# Autodesk Inventor assembly: ElectronicsLayout
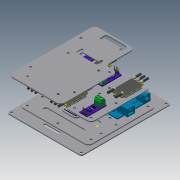
[picture p0: Inventor's stored thumbnail of the model, 180x180]
Saved by Autodesk Inventor 2018 (Build 220112000, 112)
## iProperties
Created: 2019-03-24
Part Number: ElectronicsLayout
Document SubType Name: Assembly
Designer: anirudh
Author: anirudh
## Documents named in this file (14)
- D:\Silicon Sharks\2018-2019\ElectronicsHousing\Electronics Layout\ElectronicsLayout.iam
- D:\Silicon Sharks\2018-2019\ElectronicsHousing\Electronics Layout\Tier1Plate.ipt
- C:\Users\anirudh\Documents\MARS Fund\MATE Robotics\Silicon Sharks\2018-2019\ElectronicsHousing\Electronics Layout\Hex Spacer MF M3 L6mm.ipt
- C:\Users\anirudh\Documents\MARS Fund\MATE Robotics\Silicon Sharks\2018-2019\ElectronicsHousing\Electronics Layout\Hex Spacer MF M3 L20mm.ipt
- D:\Silicon Sharks\2018-2019\ElectronicsHousing\Electronics Layout\Tier2Plate.ipt
- D:\Silicon Sharks\2018-2019\ElectronicsHousing\Electronics Layout\BESC30-R3.ipt
- D:\Silicon Sharks\2018-2019\ElectronicsHousing\Electronics Layout\ACS 712 Stromsensor für Arduino.ipt
- D:\Silicon Sharks\2018-2019\ElectronicsHousing\Electronics Layout\Tier3Plate.ipt
- D:\Silicon Sharks\2018-2019\ElectronicsHousing\Electronics Layout\PCB2x8.ipt
- D:\Silicon Sharks\2018-2019\ElectronicsHousing\Electronics Layout\ArduinoMega_STEP_AP203.ipt
- D:\Silicon Sharks\2018-2019\ElectronicsHousing\Electronics Layout\Tier4.ipt
- D:\Silicon Sharks\2018-2019\ElectronicsHousing\Electronics Layout\Adafruit_BNO055_AP214.ipt
- C:\Users\anirudh\Documents\MARS Fund\MATE Robotics\Silicon Sharks\2018-2019\ElectronicsHousing\Electronics Layout\Hex Spacer MF M3 L8mm.ipt
- D:\Silicon Sharks\2018-2019\ElectronicsHousing\Electronics Layout\Tier5.ipt
## Components (40 placed, 13 different names)
1. Tier1Plate:1 — Mate:1, Mate:2, Mate:3, Mate:4, Mate:5, Mate:6, Mate:7, Mate:8, Mate:9, Mate:10, Mate:11, Mate:12, Mate:13, Mate:14, Mate:15, Mate:16, Mate:17, Mate:18, Mate:19, Mate:20, Mate:21, Mate:22, Mate:23, Mate:24
2. Hex Spacer MF M3 L6mm:1 — Mate:1, Mate:12
3. Hex Spacer MF M3 L6mm:2 — Mate:2, Mate:13
4. Hex Spacer MF M3 L6mm:3 — Mate:4, Mate:11
5. Hex Spacer MF M3 L6mm:4 — Mate:3, Mate:14
6. Hex Spacer MF M3 L6mm:5 — Mate:7, Mate:15
7. Hex Spacer MF M3 L6mm:6 — Mate:8, Mate:9
8. Hex Spacer MF M3 L6mm:7 — Mate:5, Mate:16
9. Hex Spacer MF M3 L6mm:8 — Mate:6, Mate:10
10. Hex Spacer MF M3 L20mm:1 — Mate:18, Mate:21, Mate:26
11. Hex Spacer MF M3 L20mm:2 — Mate:17, Mate:22, Mate:25, Mate:27
12. Hex Spacer MF M3 L20mm:3 — Mate:19, Mate:23
13. Hex Spacer MF M3 L20mm:4 — Mate:20, Mate:24
14. Tier2Plate:1 — Mate:25, Mate:26, Mate:27, Mate:28, Mate:29, Mate:30, Mate:31, Mate:32, Mate:33, Mate:34, Mate:35, Mate:36, Mate:37, Mate:38, Mate:39, Flush:3, Flush:4, Flush:5, Flush:6, Flush:7, Flush:8, Flush:9, Flush:10, Flush:11, Flush:12, Flush:13, Flush:14, Flush:15, Flush:16, Flush:17, Flush:18, Mate:93, Mate:94, Mate:95
15. BESC30-R3:1 — Mate:28, Flush:5, Flush:6
16. BESC30-R3:2 — Mate:29, Flush:3, Flush:4
17. BESC30-R3:3 — Mate:30, Flush:7, Flush:8
18. BESC30-R3:4 — Mate:31, Flush:9, Flush:10
19. ACS 712 Stromsensor für Arduino:1 — Mate:33, Flush:15, Flush:17
20. ACS 712 Stromsensor für Arduino:2 — Mate:35, Flush:11, Flush:12
21. ACS 712 Stromsensor für Arduino:3 — Mate:32, Flush:16, Flush:18
22. ACS 712 Stromsensor für Arduino:4 — Mate:34, Flush:13, Flush:14
23. Hex Spacer MF M3 L6mm:9 — Mate:36, Mate:39, Mate:40, Mate:42
24. Hex Spacer MF M3 L6mm:10 — Mate:37, Mate:38, Mate:41
25. Tier3Plate:1 — Mate:40, Mate:41, Mate:42, Flush:1, Flush:2, Mate:43, Mate:64, Mate:65, Mate:66
26. PCB2x8:1 — Flush:1, Flush:2, Mate:43
27. Adafruit_BNO055_AP214:1 — Mate:64, Mate:65, Mate:66
28. Tier4:1 — Mate:67, Mate:68, Mate:69, Mate:70, Mate:71, Mate:72, Mate:73, Mate:77, Mate:87, Mate:88, Mate:89, Mate:90, Mate:91, Mate:92, Mate:96, Flush:19, Flush:20
29. Hex Spacer MF M3 L6mm:11 — Mate:69, Mate:71, Mate:75, Mate:76
30. Hex Spacer MF M3 L6mm:12 — Mate:70, Mate:72, Mate:80
31. Hex Spacer MF M3 L6mm:13 — Mate:67, Mate:73, Mate:79
32. Hex Spacer MF M3 L6mm:14 — Mate:68, Mate:77, Mate:78
33. ArduinoMega_STEP_AP203:1 — Mate:75, Mate:76, Mate:78, Mate:79, Mate:80
34. Hex Spacer MF M3 L8mm:1 — Mate:85, Mate:86, Mate:90, Mate:93
35. Hex Spacer MF M3 L20mm:5 — Mate:85, Mate:86, Mate:87
36. Hex Spacer MF M3 L8mm:2 — Mate:83, Mate:84, Mate:91, Mate:94
37. Hex Spacer MF M3 L20mm:6 — Mate:83, Mate:84, Mate:88
38. Hex Spacer MF M3 L8mm:3 — Mate:81, Mate:82, Mate:92, Mate:95
39. Hex Spacer MF M3 L20mm:7 — Mate:81, Mate:82, Mate:89
40. Tier5:1 — Mate:96, Flush:19, Flush:20
## Relationships (95: Mate 75, Flush 20)
- Mate:1: Tier1Plate:1 ↔ Hex Spacer MF M3 L6mm:1
- Mate:2: Tier1Plate:1 ↔ Hex Spacer MF M3 L6mm:2
- Mate:3: Tier1Plate:1 ↔ Hex Spacer MF M3 L6mm:4
- Mate:4: Tier1Plate:1 ↔ Hex Spacer MF M3 L6mm:3
- Mate:5: Tier1Plate:1 ↔ Hex Spacer MF M3 L6mm:7
- Mate:6: Tier1Plate:1 ↔ Hex Spacer MF M3 L6mm:8
- Mate:7: Tier1Plate:1 ↔ Hex Spacer MF M3 L6mm:5
- Mate:8: Tier1Plate:1 ↔ Hex Spacer MF M3 L6mm:6
- Mate:9: Tier1Plate:1 ↔ Hex Spacer MF M3 L6mm:6
- Mate:10: Tier1Plate:1 ↔ Hex Spacer MF M3 L6mm:8
- Mate:11: Tier1Plate:1 ↔ Hex Spacer MF M3 L6mm:3
- Mate:12: Tier1Plate:1 ↔ Hex Spacer MF M3 L6mm:1
- Mate:13: Tier1Plate:1 ↔ Hex Spacer MF M3 L6mm:2
- Mate:14: Tier1Plate:1 ↔ Hex Spacer MF M3 L6mm:4
- Mate:15: Tier1Plate:1 ↔ Hex Spacer MF M3 L6mm:5
- Mate:16: Tier1Plate:1 ↔ Hex Spacer MF M3 L6mm:7
- Mate:17: Tier1Plate:1 ↔ Hex Spacer MF M3 L20mm:2
- Mate:18: Tier1Plate:1 ↔ Hex Spacer MF M3 L20mm:1
- Mate:19: Tier1Plate:1 ↔ Hex Spacer MF M3 L20mm:3
- Mate:20: Tier1Plate:1 ↔ Hex Spacer MF M3 L20mm:4
- Mate:21: Tier1Plate:1 ↔ Hex Spacer MF M3 L20mm:1
- Mate:22: Tier1Plate:1 ↔ Hex Spacer MF M3 L20mm:2
- Mate:23: Tier1Plate:1 ↔ Hex Spacer MF M3 L20mm:3
- Mate:24: Tier1Plate:1 ↔ Hex Spacer MF M3 L20mm:4
- Mate:25: Hex Spacer MF M3 L20mm:2 ↔ Tier2Plate:1
- Mate:26: Hex Spacer MF M3 L20mm:1 ↔ Tier2Plate:1
- Mate:27: Hex Spacer MF M3 L20mm:2 ↔ Tier2Plate:1
- Mate:28: Tier2Plate:1 ↔ BESC30-R3:1
- Mate:29: Tier2Plate:1 ↔ BESC30-R3:2
- Mate:30: Tier2Plate:1 ↔ BESC30-R3:3
- Mate:31: Tier2Plate:1 ↔ BESC30-R3:4
- Mate:32: Tier2Plate:1 ↔ ACS 712 Stromsensor für Arduino:3
- Mate:33: Tier2Plate:1 ↔ ACS 712 Stromsensor für Arduino:1
- Mate:34: Tier2Plate:1 ↔ ACS 712 Stromsensor für Arduino:4
- Mate:35: Tier2Plate:1 ↔ ACS 712 Stromsensor für Arduino:2
- Mate:36: Tier2Plate:1 ↔ Hex Spacer MF M3 L6mm:9
- Mate:37: Tier2Plate:1 ↔ Hex Spacer MF M3 L6mm:10
- Mate:38: Tier2Plate:1 ↔ Hex Spacer MF M3 L6mm:10
- Mate:39: Tier2Plate:1 ↔ Hex Spacer MF M3 L6mm:9
- Mate:40: Hex Spacer MF M3 L6mm:9 ↔ Tier3Plate:1
- Mate:41: Hex Spacer MF M3 L6mm:10 ↔ Tier3Plate:1
- Mate:42: Hex Spacer MF M3 L6mm:9 ↔ Tier3Plate:1
- Flush:1 (-2.6797 mm): Tier3Plate:1 ↔ PCB2x8:1
- Flush:2 (1.1557 mm): Tier3Plate:1 ↔ PCB2x8:1
- Flush:3: Tier2Plate:1 ↔ BESC30-R3:2
- Flush:4: Tier2Plate:1 ↔ BESC30-R3:2
- Flush:5: Tier2Plate:1 ↔ BESC30-R3:1
- Flush:6: Tier2Plate:1 ↔ BESC30-R3:1
- Flush:7: Tier2Plate:1 ↔ BESC30-R3:3
- Flush:8: Tier2Plate:1 ↔ BESC30-R3:3
- Flush:9: Tier2Plate:1 ↔ BESC30-R3:4
- Flush:10: Tier2Plate:1 ↔ BESC30-R3:4
- Flush:11 (1.7272 mm): Tier2Plate:1 ↔ ACS 712 Stromsensor für Arduino:2
- Flush:12 (3.8862 mm): Tier2Plate:1 ↔ ACS 712 Stromsensor für Arduino:2
- Flush:13 (3.8862 mm): Tier2Plate:1 ↔ ACS 712 Stromsensor für Arduino:4
- Flush:14 (10.0838 mm): Tier2Plate:1 ↔ ACS 712 Stromsensor für Arduino:4
- Flush:15 (3.8862 mm): Tier2Plate:1 ↔ ACS 712 Stromsensor für Arduino:1
- Flush:16 (3.8862 mm): Tier2Plate:1 ↔ ACS 712 Stromsensor für Arduino:3
- Flush:17 (4.699 mm): Tier2Plate:1 ↔ ACS 712 Stromsensor für Arduino:1
- Flush:18 (4.699 mm): Tier2Plate:1 ↔ ACS 712 Stromsensor für Arduino:3
- Mate:43: Tier3Plate:1 ↔ PCB2x8:1
- Mate:64: Tier3Plate:1 ↔ Adafruit_BNO055_AP214:1
- Mate:65: Tier3Plate:1 ↔ Adafruit_BNO055_AP214:1
- Mate:66: Tier3Plate:1 ↔ Adafruit_BNO055_AP214:1
- Mate:67: Tier4:1 ↔ Hex Spacer MF M3 L6mm:13
- Mate:68: Tier4:1 ↔ Hex Spacer MF M3 L6mm:14
- Mate:69: Tier4:1 ↔ Hex Spacer MF M3 L6mm:11
- Mate:70: Tier4:1 ↔ Hex Spacer MF M3 L6mm:12
- Mate:71: Tier4:1 ↔ Hex Spacer MF M3 L6mm:11
- Mate:72: Tier4:1 ↔ Hex Spacer MF M3 L6mm:12
- Mate:73: Tier4:1 ↔ Hex Spacer MF M3 L6mm:13
- Mate:75: Hex Spacer MF M3 L6mm:11 ↔ ArduinoMega_STEP_AP203:1
- Mate:76: Hex Spacer MF M3 L6mm:11 ↔ ArduinoMega_STEP_AP203:1
- Mate:77: Tier4:1 ↔ Hex Spacer MF M3 L6mm:14
- Mate:78: Hex Spacer MF M3 L6mm:14 ↔ ArduinoMega_STEP_AP203:1
- Mate:79: Hex Spacer MF M3 L6mm:13 ↔ ArduinoMega_STEP_AP203:1
- Mate:80: Hex Spacer MF M3 L6mm:12 ↔ ArduinoMega_STEP_AP203:1
- Mate:81: Hex Spacer MF M3 L8mm:3 ↔ Hex Spacer MF M3 L20mm:7
- Mate:82: Hex Spacer MF M3 L8mm:3 ↔ Hex Spacer MF M3 L20mm:7
- Mate:83: Hex Spacer MF M3 L8mm:2 ↔ Hex Spacer MF M3 L20mm:6
- Mate:84: Hex Spacer MF M3 L8mm:2 ↔ Hex Spacer MF M3 L20mm:6
- Mate:85: Hex Spacer MF M3 L8mm:1 ↔ Hex Spacer MF M3 L20mm:5
- Mate:86: Hex Spacer MF M3 L8mm:1 ↔ Hex Spacer MF M3 L20mm:5
- Mate:87: Tier4:1 ↔ Hex Spacer MF M3 L20mm:5
- Mate:88: Tier4:1 ↔ Hex Spacer MF M3 L20mm:6
- Mate:89: Tier4:1 ↔ Hex Spacer MF M3 L20mm:7
- Mate:90: Tier4:1 ↔ Hex Spacer MF M3 L8mm:1
- Mate:91: Tier4:1 ↔ Hex Spacer MF M3 L8mm:2
- Mate:92: Tier4:1 ↔ Hex Spacer MF M3 L8mm:3
- Mate:93: Tier2Plate:1 ↔ Hex Spacer MF M3 L8mm:1
- Mate:94: Tier2Plate:1 ↔ Hex Spacer MF M3 L8mm:2
- Mate:95: Tier2Plate:1 ↔ Hex Spacer MF M3 L8mm:3
- Mate:96 (0.9398 mm): Tier4:1 ↔ Tier5:1
- Flush:19 (-16.4592 mm): Tier4:1 ↔ Tier5:1
- Flush:20 (-5.2578 mm): Tier4:1 ↔ Tier5:1
